# Autodesk Inventor assembly: Overall_Assembly
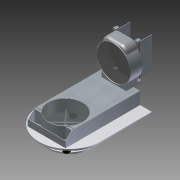
[picture p0: Inventor's stored thumbnail of the model, 180x180]
Saved by Autodesk Inventor 2011 SP1 (Build 150282100, 282)
## iProperties
Created: 2011-06-12
Part Number: Overall_Assembly
Document SubType Name: Assembly
Designer: Andrew G. Meyer
Mass: 4389.74 g
Surface Area: 19725.4 cm^2
Volume: 4389.74 cm^3
Density: 1 g/cm^3
Author: Andrew G. Meyer
## Documents named in this file (6)
- C:\Users\Andrew G. Meyer\Documents\Inventor\Hovercraft\Overall_Assembly.iam
- C:\Users\Andrew G. Meyer\Documents\Inventor\Hovercraft\Bottom_Deck.ipt
- C:\Users\Andrew G. Meyer\Documents\Inventor\Hovercraft\Deck_Bolt.ipt
- C:\Users\Andrew G. Meyer\Documents\Inventor\Hovercraft\Deck_Spacer.ipt
- C:\Users\Andrew G. Meyer\Documents\Inventor\Hovercraft\Top_Deck.ipt
- C:\Users\Andrew G. Meyer\Documents\Inventor\Hovercraft\Upper_Deck.iam
## Components (15 placed, 5 different names)
1. Bottom_Deck:1 — Insert:1, Insert:2, Insert:3, Insert:4, Insert:5, Insert:6
2. Deck_Bolt:1 — Insert:4, Insert:10
3. Deck_Bolt:2 — Insert:5, Insert:11
4. Deck_Bolt:3 — Insert:6, Insert:12
5. Deck_Bolt:4 — Insert:3, Insert:9
6. Deck_Bolt:5 — Insert:2, Insert:8
7. Deck_Bolt:6 — Insert:1, Insert:7
8. Deck_Spacer:1 — Insert:12
9. Deck_Spacer:2 — Insert:11
10. Deck_Spacer:3 — Insert:10
11. Deck_Spacer:4 — Insert:8, Insert:14
12. Deck_Spacer:5 — Insert:7, Insert:13
13. Deck_Spacer:6 — Insert:9
14. Top_Deck:1 — Insert:13, Insert:14, Insert:15, Insert:16
15. Upper_Deck:1 [sub-assembly] — Insert:15, Insert:16
## Relationships (16: Insert 16)
- Insert:1: Bottom_Deck:1 ↔ Deck_Bolt:6
- Insert:2: Bottom_Deck:1 ↔ Deck_Bolt:5
- Insert:3: Bottom_Deck:1 ↔ Deck_Bolt:4
- Insert:4: Bottom_Deck:1 ↔ Deck_Bolt:1
- Insert:5: Bottom_Deck:1 ↔ Deck_Bolt:2
- Insert:6: Bottom_Deck:1 ↔ Deck_Bolt:3
- Insert:7 (9.525 mm): Deck_Bolt:6 ↔ Deck_Spacer:5
- Insert:8 (9.525 mm): Deck_Bolt:5 ↔ Deck_Spacer:4
- Insert:9 (9.525 mm): Deck_Bolt:4 ↔ Deck_Spacer:6
- Insert:10 (9.525 mm): Deck_Bolt:1 ↔ Deck_Spacer:3
- Insert:11 (9.525 mm): Deck_Bolt:2 ↔ Deck_Spacer:2
- Insert:12 (9.525 mm): Deck_Bolt:3 ↔ Deck_Spacer:1
- Insert:13: Deck_Spacer:5 ↔ Top_Deck:1
- Insert:14: Deck_Spacer:4 ↔ Top_Deck:1
- Insert:15: Top_Deck:1 ↔ Upper_Deck:1
- Insert:16: Top_Deck:1 ↔ Upper_Deck:1
